# Autodesk Inventor assembly: SPE1V1 Estructura
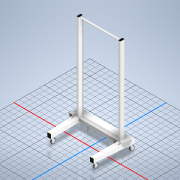
[picture p0: Inventor's stored thumbnail of the model, 180x180]
Saved by Autodesk Inventor 2021.2 (Build 252289000, 289)
## iProperties
Created: 2026-06-02
Part Number: SPE1V1 Estructura
Document SubType Name: Assembly
Designer: nelso
Author: nelso
## Documents named in this file (24)
- C:\Users\nelso\Documents\Escritorio\Soporte-Paciente-Espinografia\Workspace\SPE1V1 Estructura.iam
- C:\Users\nelso\Documents\Escritorio\Soporte-Paciente-Espinografia\Workspace\SP22V1 Tubo 40x80x1825mm.ipt
- C:\Users\nelso\Documents\Escritorio\Soporte-Paciente-Espinografia\Workspace\SP21V1 Tubo 40x80x100mm.ipt
- C:\Users\nelso\Documents\Escritorio\Soporte-Paciente-Espinografia\Workspace\SP23V1 Cobertora Derecha.ipt
- C:\Users\nelso\Documents\Escritorio\Soporte-Paciente-Espinografia\Workspace\SP24V1 Cobertora Izquierda.ipt
- C:\Users\nelso\Documents\Escritorio\Soporte-Paciente-Espinografia\Workspace\SP20V1 Tubo 80x120x790mm.ipt
- C:\Users\nelso\Documents\Escritorio\Soporte-Paciente-Espinografia\Workspace\SP19V1 Tapacanto Delantero.ipt
- C:\Users\nelso\Documents\Escritorio\Soporte-Paciente-Espinografia\Workspace\SP18V1 Tapacanto Superior.ipt
- C:\Users\nelso\Documents\Escritorio\Soporte-Paciente-Espinografia\Workspace\RFPLUS8PO300.ipt
- C:\Users\nelso\Documents\Escritorio\Soporte-Paciente-Espinografia\Workspace\SP17V1 Varilla Pedal.ipt
- C:\Users\nelso\Documents\Escritorio\Soporte-Paciente-Espinografia\Workspace\SP16V1 Buje Pedal.ipt
- C:\Users\nelso\Documents\Escritorio\Soporte-Paciente-Espinografia\Workspace\SP15V1 Pedal Izquierdo.ipt
- C:\Users\nelso\Documents\Escritorio\Soporte-Paciente-Espinografia\Workspace\SPE3V1 Freno.iam
- C:\Users\nelso\Documents\Escritorio\Soporte-Paciente-Espinografia\Workspace\SP14V1 Pedal Derecho.ipt
- C:\Users\nelso\Documents\Escritorio\Soporte-Paciente-Espinografia\Workspace\G3-100-PPP-RU.ipt
- C:\Users\nelso\Documents\Escritorio\Soporte-Paciente-Espinografia\Workspace\SP33V1 Tope Base.ipt
- C:\Users\nelso\Documents\Escritorio\Soporte-Paciente-Espinografia\Workspace\SP38V1 Cobertor Freno.ipt
- C:\Users\nelso\Documents\Escritorio\Soporte-Paciente-Espinografia\Workspace\SP43V1 Tubo 40x80x1825mm.ipt
- C:\Users\nelso\Documents\Escritorio\Soporte-Paciente-Espinografia\Workspace\DIN 555A10C.ipt
- C:\Users\nelso\Documents\Escritorio\Soporte-Paciente-Espinografia\Workspace\DIN125-A8,4C.ipt
- C:\Users\nelso\Documents\Escritorio\Soporte-Paciente-Espinografia\Workspace\DIN933M8X1.25L20C.ipt
- C:\Users\nelso\Documents\Escritorio\Soporte-Paciente-Espinografia\Workspace\SP11V1 Planchuela Baranda.ipt
- C:\Users\nelso\Documents\Escritorio\Soporte-Paciente-Espinografia\Workspace\SP52V1 Tubo superior.ipt
- C:\Users\nelso\Documents\Escritorio\Soporte-Paciente-Espinografia\Workspace\SP55V1 Chapa Guia.ipt
## Components (59 placed, 23 different names)
1. SP43V1 Tubo 40x80x1825mm:1 — Nivelación:17, Coincidencia:54, Coincidencia:55, Coincidencia:68, Nivelación:67, Coincidencia:71, Flush:75, Flush:76, Flush:77, Flush:78, Flush:79, Mate:84, Mate:85, Mate:86, Mate:87, Mate:88, Mate:107, Flush:101, Mate:235, Flush:149, Flush:150, Mate:238, Mate:239, Mate:242, Mate:246, Mate:247
2. SP18V1 Tapacanto Superior:1 — Coincidencia:68, Nivelación:67, Coincidencia:71
3. SP22V1 Tubo 40x80x1825mm:2 — Mate:179, Mate:180, Flush:120, Mate:181, Mate:182, Mate:183, Mate:184, Mate:185, Mate:186, Mate:187, Flush:121, Flush:122, Flush:123, Flush:124, Flush:125, Flush:126, Mate:222, Flush:145, Flush:146, Mate:236, Mate:237, Mate:243, Mate:244, Mate:245
4. SP18V1 Tapacanto Superior:2 — Mate:181
5. SP21V1 Tubo 40x80x100mm:1 — Nivelación:14, Coincidencia:24, Coincidencia:42, Mate:203, Mate:204, Flush:134
6. SP19V1 Tapacanto Delantero:1 — Mate:208, Flush:141, Flush:142
7. SP21V1 Tubo 40x80x100mm:2 — Coincidencia:37, Coincidencia:38, Coincidencia:66, Mate:206, Flush:136, Mate:207
8. SP21V1 Tubo 40x80x100mm:3 — Coincidencia:50, Coincidencia:51, Coincidencia:65, Mate:158, Mate:205, Flush:135
9. SP21V1 Tubo 40x80x100mm:4 — Mate:150, Mate:151, Mate:201, Mate:202, Flush:133
10. SP19V1 Tapacanto Delantero:2 — Flush:139, Flush:140, Mate:213
11. SP23V1 Cobertora Derecha:1 — Nivelación:14, Coincidencia:24, Nivelación:17, Coincidencia:37, Coincidencia:38, Nivelación:18, Coincidencia:42, Coincidencia:55, Nivelación:27, Coincidencia:66, Flush:105, Mate:126, Mate:131, Mate:174, Flush:118, Mate:194, Mate:195, Mate:196, Mate:197, Flush:131, Mate:208, Mate:210, Mate:212, Flush:141, Flush:142
12. SP24V1 Cobertora Izquierda:1 — Nivelación:18, Coincidencia:50, Coincidencia:51, Nivelación:24, Nivelación:28, Coincidencia:65, Flush:104, Mate:127, Mate:150, Mate:151, Mate:180, Flush:120, Mate:192, Mate:193, Mate:198, Mate:199, Flush:129, Mate:209, Flush:139, Flush:140, Mate:213
13. SP20V1 Tubo 80x120x790mm:1 — Nivelación:24, Coincidencia:54, Nivelación:27, Nivelación:28, Mate:110, Mate:111, Mate:124, Flush:119, Mate:177, Mate:179, Flush:127, Flush:137, Mate:209, Mate:210, Mate:211
14. RFPLUS8PO300:1 — Mate:107, Flush:101
15. RFPLUS8PO300:2 — Flush:75, Mate:88
16. RFPLUS8PO300:3 — Flush:76, Mate:87
17. RFPLUS8PO300:4 — Flush:77, Mate:86
18. RFPLUS8PO300:5 — Flush:78, Mate:84
19. RFPLUS8PO300:6 — Flush:79, Mate:85
20. SP17V1 Varilla Pedal:1 — Mate:117, Mate:118, Mate:119, Mate:120, Mate:121, Mate:125, Mate:128, Mate:129, Mate:130, Mate:132, Mate:133, Mate:134, Flush:127
21. SP16V1 Buje Pedal:1 — Mate:116, Flush:105, Mate:131
22. SP16V1 Buje Pedal:2 — Mate:116, Mate:125, Flush:104
23. SP14V1 Pedal Derecho:1 — Mate:128, Mate:129, Mate:130, Mate:132, Mate:200
24. SP15V1 Pedal Izquierdo:1 — Mate:120, Mate:121, Flush:132
25. SPE3V1 Freno:1 [sub-assembly] — Mate:110, Flush:103, Mate:117, Mate:118, Mate:119, Mate:124, Mate:127
26. SPE3V1 Freno:2 [sub-assembly] — Mate:111, Flush:103, Mate:126, Mate:133, Mate:134
27. RFPLUS8PO300:17 — Mate:187, Flush:121
28. RFPLUS8PO300:18 — Mate:186, Flush:122
29. RFPLUS8PO300:19 — Mate:185, Flush:123
30. RFPLUS8PO300:20 — Mate:184, Flush:124
31. RFPLUS8PO300:21 — Mate:182, Flush:125
32. RFPLUS8PO300:22 — Mate:183, Flush:126
33. G3-100-PPP-RU:1 — Mate:206, Flush:136, Mate:207
34. G3-100-PPP-RU:2 — Mate:203, Mate:204, Flush:134
35. G3-100-PPP-RU:3 — Mate:201, Mate:202, Flush:133
36. G3-100-PPP-RU:4 — Mate:158, Mate:205, Flush:135
37. SP33V1 Tope Base:1 — Mate:174, Flush:118, Mate:178
38. SP38V1 Cobertor Freno:1 — Flush:119, Mate:177, Mate:178, Flush:138
39. DIN 555A10C:1 — Mate:195, Mate:196
40. DIN 555A10C:2 — Mate:194, Mate:197
41. DIN 555A10C:3 — Mate:192, Mate:198
42. DIN 555A10C:4 — Mate:193, Mate:199
43. DIN125-A8,4C:1 — Mate:214, Mate:215, Mate:219
44. DIN933M8X1.25L20C:1 — Mate:214, Mate:215, Mate:220, Mate:224, Mate:236
45. SP11V1 Planchuela Baranda:1 — Mate:218, Mate:219, Mate:220, Mate:221, Mate:222
46. DIN125-A8,4C:2 — Mate:216, Mate:217, Mate:218
47. DIN933M8X1.25L20C:2 — Mate:216, Mate:217, Mate:221, Mate:223, Mate:237
48. RFPLUS8PO300:23 — Flush:146, Mate:223
49. RFPLUS8PO300:24 — Flush:145, Mate:224
50. DIN125-A8,4C:3
51. DIN933M8X1.25L20C:3 — Mate:238
52. SP11V1 Planchuela Baranda:2 — Mate:235, Mate:241
53. DIN125-A8,4C:4
54. DIN933M8X1.25L20C:4 — Mate:239
55. RFPLUS8PO300:25 — Flush:150
56. RFPLUS8PO300:26 — Flush:149
57. SP52V1 Tubo superior:1 — Mate:240, Mate:241
58. SP55V1 Chapa Guia:1 — Mate:243, Mate:244, Mate:245
59. SP55V1 Chapa Guia:2 — Mate:242, Mate:246, Mate:247
## Relationships (153: Mate 109, Flush 44)
- Nivelación:14 [Flush]: SP21V1 Tubo 40x80x100mm:1 ↔ SP23V1 Cobertora Derecha:1
- Coincidencia:24 [Mate] (0.5 mm): SP21V1 Tubo 40x80x100mm:1 ↔ SP23V1 Cobertora Derecha:1
- Nivelación:17 [Flush]: SP43V1 Tubo 40x80x1825mm:1 ↔ SP23V1 Cobertora Derecha:1
- Coincidencia:37 [Mate]: SP21V1 Tubo 40x80x100mm:2 ↔ SP23V1 Cobertora Derecha:1
- Coincidencia:38 [Mate]: SP21V1 Tubo 40x80x100mm:2 ↔ SP23V1 Cobertora Derecha:1
- Nivelación:18 [Flush]: SP23V1 Cobertora Derecha:1 ↔ SP24V1 Cobertora Izquierda:1
- Coincidencia:42 [Mate]: SP21V1 Tubo 40x80x100mm:1 ↔ SP23V1 Cobertora Derecha:1
- Coincidencia:50 [Mate]: SP21V1 Tubo 40x80x100mm:3 ↔ SP24V1 Cobertora Izquierda:1
- Coincidencia:51 [Mate]: SP21V1 Tubo 40x80x100mm:3 ↔ SP24V1 Cobertora Izquierda:1
- Nivelación:24 [Flush]: SP24V1 Cobertora Izquierda:1 ↔ SP20V1 Tubo 80x120x790mm:1
- Coincidencia:54 [Mate]: SP43V1 Tubo 40x80x1825mm:1 ↔ SP20V1 Tubo 80x120x790mm:1
- Coincidencia:55 [Mate]: SP43V1 Tubo 40x80x1825mm:1 ↔ SP23V1 Cobertora Derecha:1
- Nivelación:27 [Flush]: SP23V1 Cobertora Derecha:1 ↔ SP20V1 Tubo 80x120x790mm:1
- Nivelación:28 [Flush]: SP24V1 Cobertora Izquierda:1 ↔ SP20V1 Tubo 80x120x790mm:1
- Coincidencia:65 [Mate]: SP21V1 Tubo 40x80x100mm:3 ↔ SP24V1 Cobertora Izquierda:1
- Coincidencia:66 [Mate]: SP21V1 Tubo 40x80x100mm:2 ↔ SP23V1 Cobertora Derecha:1
- Coincidencia:68 [Mate]: SP43V1 Tubo 40x80x1825mm:1 ↔ SP18V1 Tapacanto Superior:1
- Nivelación:67 [Flush]: SP43V1 Tubo 40x80x1825mm:1 ↔ SP18V1 Tapacanto Superior:1
- Coincidencia:71 [Mate]: SP43V1 Tubo 40x80x1825mm:1 ↔ SP18V1 Tapacanto Superior:1
- Flush:75: SP43V1 Tubo 40x80x1825mm:1 ↔ RFPLUS8PO300:2
- Flush:76: SP43V1 Tubo 40x80x1825mm:1 ↔ RFPLUS8PO300:3
- Flush:77: SP43V1 Tubo 40x80x1825mm:1 ↔ RFPLUS8PO300:4
- Flush:78: SP43V1 Tubo 40x80x1825mm:1 ↔ RFPLUS8PO300:5
- Flush:79: SP43V1 Tubo 40x80x1825mm:1 ↔ RFPLUS8PO300:6
- Mate:84: SP43V1 Tubo 40x80x1825mm:1 ↔ RFPLUS8PO300:5
- Mate:85: SP43V1 Tubo 40x80x1825mm:1 ↔ RFPLUS8PO300:6
- Mate:86: SP43V1 Tubo 40x80x1825mm:1 ↔ RFPLUS8PO300:4
- Mate:87: SP43V1 Tubo 40x80x1825mm:1 ↔ RFPLUS8PO300:3
- Mate:88: SP43V1 Tubo 40x80x1825mm:1 ↔ RFPLUS8PO300:2
- Mate:107: SP43V1 Tubo 40x80x1825mm:1 ↔ RFPLUS8PO300:1
- Flush:101: SP43V1 Tubo 40x80x1825mm:1 ↔ RFPLUS8PO300:1
- Mate:110: SP20V1 Tubo 80x120x790mm:1 ↔ SPE3V1 Freno:1
- Mate:111: SP20V1 Tubo 80x120x790mm:1 ↔ SPE3V1 Freno:2
- Mate:116: SP16V1 Buje Pedal:1 ↔ SP16V1 Buje Pedal:2
- Flush:103: SPE3V1 Freno:1 ↔ SPE3V1 Freno:2
- Mate:117: SP17V1 Varilla Pedal:1 ↔ SPE3V1 Freno:1
- Mate:118: SP17V1 Varilla Pedal:1 ↔ SPE3V1 Freno:1
- Mate:119: SP17V1 Varilla Pedal:1 ↔ SPE3V1 Freno:1
- Mate:120: SP17V1 Varilla Pedal:1 ↔ SP15V1 Pedal Izquierdo:1
- Mate:121: SP17V1 Varilla Pedal:1 ↔ SP15V1 Pedal Izquierdo:1
- Mate:124: SP20V1 Tubo 80x120x790mm:1 ↔ SPE3V1 Freno:1
- Mate:125: SP17V1 Varilla Pedal:1 ↔ SP16V1 Buje Pedal:2
- Flush:104: SP24V1 Cobertora Izquierda:1 ↔ SP16V1 Buje Pedal:2
- Flush:105: SP23V1 Cobertora Derecha:1 ↔ SP16V1 Buje Pedal:1
- Mate:126 (100 mm): SP23V1 Cobertora Derecha:1 ↔ SPE3V1 Freno:2
- Mate:127 (100 mm): SP24V1 Cobertora Izquierda:1 ↔ SPE3V1 Freno:1
- Mate:128: SP17V1 Varilla Pedal:1 ↔ SP14V1 Pedal Derecho:1
- Mate:129: SP17V1 Varilla Pedal:1 ↔ SP14V1 Pedal Derecho:1
- Mate:130: SP17V1 Varilla Pedal:1 ↔ SP14V1 Pedal Derecho:1
- Mate:131: SP23V1 Cobertora Derecha:1 ↔ SP16V1 Buje Pedal:1
- Mate:132: SP17V1 Varilla Pedal:1 ↔ SP14V1 Pedal Derecho:1
- Mate:133: SP17V1 Varilla Pedal:1 ↔ SPE3V1 Freno:2
- Mate:134: SP17V1 Varilla Pedal:1 ↔ SPE3V1 Freno:2
- [Flush]: SP22V1 Tubo 40x80x1825mm:2 ↔ SP18V1 Tapacanto Superior:2
- [Mate]: SP22V1 Tubo 40x80x1825mm:2 ↔ SP18V1 Tapacanto Superior:2
- Mate:150 (0.5 mm): SP21V1 Tubo 40x80x100mm:4 ↔ SP24V1 Cobertora Izquierda:1
- Mate:151: SP21V1 Tubo 40x80x100mm:4 ↔ SP24V1 Cobertora Izquierda:1
- Mate:158: SP21V1 Tubo 40x80x100mm:3 ↔ G3-100-PPP-RU:4
- Mate:174: SP23V1 Cobertora Derecha:1 ↔ SP33V1 Tope Base:1
- Flush:118: SP23V1 Cobertora Derecha:1 ↔ SP33V1 Tope Base:1
- Flush:119: SP20V1 Tubo 80x120x790mm:1 ↔ SP38V1 Cobertor Freno:1
- Mate:177: SP20V1 Tubo 80x120x790mm:1 ↔ SP38V1 Cobertor Freno:1
- Mate:178: SP33V1 Tope Base:1 ↔ SP38V1 Cobertor Freno:1
- Mate:179: SP22V1 Tubo 40x80x1825mm:2 ↔ SP20V1 Tubo 80x120x790mm:1
- Mate:180: SP22V1 Tubo 40x80x1825mm:2 ↔ SP24V1 Cobertora Izquierda:1
- Flush:120: SP22V1 Tubo 40x80x1825mm:2 ↔ SP24V1 Cobertora Izquierda:1
- Mate:181: SP22V1 Tubo 40x80x1825mm:2 ↔ SP18V1 Tapacanto Superior:2
- Mate:182: SP22V1 Tubo 40x80x1825mm:2 ↔ RFPLUS8PO300:21
- Mate:183: SP22V1 Tubo 40x80x1825mm:2 ↔ RFPLUS8PO300:22
- Mate:184: SP22V1 Tubo 40x80x1825mm:2 ↔ RFPLUS8PO300:20
- Mate:185: SP22V1 Tubo 40x80x1825mm:2 ↔ RFPLUS8PO300:19
- Mate:186: SP22V1 Tubo 40x80x1825mm:2 ↔ RFPLUS8PO300:18
- Mate:187: SP22V1 Tubo 40x80x1825mm:2 ↔ RFPLUS8PO300:17
- Flush:121: SP22V1 Tubo 40x80x1825mm:2 ↔ RFPLUS8PO300:17
- Flush:122: SP22V1 Tubo 40x80x1825mm:2 ↔ RFPLUS8PO300:18
- Flush:123: SP22V1 Tubo 40x80x1825mm:2 ↔ RFPLUS8PO300:19
- Flush:124: SP22V1 Tubo 40x80x1825mm:2 ↔ RFPLUS8PO300:20
- Flush:125: SP22V1 Tubo 40x80x1825mm:2 ↔ RFPLUS8PO300:21
- Flush:126: SP22V1 Tubo 40x80x1825mm:2 ↔ RFPLUS8PO300:22
- Mate:192: SP24V1 Cobertora Izquierda:1 ↔ DIN 555A10C:3
- Mate:193: SP24V1 Cobertora Izquierda:1 ↔ DIN 555A10C:4
- Mate:194: SP23V1 Cobertora Derecha:1 ↔ DIN 555A10C:2
- Mate:195: SP23V1 Cobertora Derecha:1 ↔ DIN 555A10C:1
- Mate:196: SP23V1 Cobertora Derecha:1 ↔ DIN 555A10C:1
- Mate:197: SP23V1 Cobertora Derecha:1 ↔ DIN 555A10C:2
- Mate:198: SP24V1 Cobertora Izquierda:1 ↔ DIN 555A10C:3
- Mate:199: SP24V1 Cobertora Izquierda:1 ↔ DIN 555A10C:4
- Flush:127: SP20V1 Tubo 80x120x790mm:1 ↔ SP17V1 Varilla Pedal:1
- Flush:129 (7.5 mm): SP24V1 Cobertora Izquierda:1
- Flush:131 (7.5 mm): SP23V1 Cobertora Derecha:1
- Flush:132: SP15V1 Pedal Izquierdo:1
- Mate:200: SP14V1 Pedal Derecho:1
- Mate:201: SP21V1 Tubo 40x80x100mm:4 ↔ G3-100-PPP-RU:3
- Mate:202: SP21V1 Tubo 40x80x100mm:4 ↔ G3-100-PPP-RU:3
- Flush:133: SP21V1 Tubo 40x80x100mm:4 ↔ G3-100-PPP-RU:3
- Mate:203: SP21V1 Tubo 40x80x100mm:1 ↔ G3-100-PPP-RU:2
- Mate:204: SP21V1 Tubo 40x80x100mm:1 ↔ G3-100-PPP-RU:2
- Flush:134: SP21V1 Tubo 40x80x100mm:1 ↔ G3-100-PPP-RU:2
- Mate:205: SP21V1 Tubo 40x80x100mm:3 ↔ G3-100-PPP-RU:4
- Flush:135: SP21V1 Tubo 40x80x100mm:3 ↔ G3-100-PPP-RU:4
- Mate:206: SP21V1 Tubo 40x80x100mm:2 ↔ G3-100-PPP-RU:1
- Flush:136: SP21V1 Tubo 40x80x100mm:2 ↔ G3-100-PPP-RU:1
- Mate:207: SP21V1 Tubo 40x80x100mm:2 ↔ G3-100-PPP-RU:1
- Mate:208: SP19V1 Tapacanto Delantero:1 ↔ SP23V1 Cobertora Derecha:1
- Flush:137: SP20V1 Tubo 80x120x790mm:1
- Mate:209: SP24V1 Cobertora Izquierda:1 ↔ SP20V1 Tubo 80x120x790mm:1
- Mate:210: SP23V1 Cobertora Derecha:1 ↔ SP20V1 Tubo 80x120x790mm:1
- Mate:211: SP20V1 Tubo 80x120x790mm:1
- Flush:138: SP38V1 Cobertor Freno:1
- Mate:212 (380 mm): SP23V1 Cobertora Derecha:1
- Flush:139: SP19V1 Tapacanto Delantero:2 ↔ SP24V1 Cobertora Izquierda:1
- Flush:140: SP19V1 Tapacanto Delantero:2 ↔ SP24V1 Cobertora Izquierda:1
- Mate:213: SP19V1 Tapacanto Delantero:2 ↔ SP24V1 Cobertora Izquierda:1
- Flush:141: SP19V1 Tapacanto Delantero:1 ↔ SP23V1 Cobertora Derecha:1
- Flush:142: SP19V1 Tapacanto Delantero:1 ↔ SP23V1 Cobertora Derecha:1
- Mate:214: DIN125-A8,4C:1 ↔ DIN933M8X1.25L20C:1
- Mate:215: DIN125-A8,4C:1 ↔ DIN933M8X1.25L20C:1
- Mate:216: DIN125-A8,4C:2 ↔ DIN933M8X1.25L20C:2
- Mate:217: DIN125-A8,4C:2 ↔ DIN933M8X1.25L20C:2
- Mate:218: SP11V1 Planchuela Baranda:1 ↔ DIN125-A8,4C:2
- Mate:219: DIN125-A8,4C:1 ↔ SP11V1 Planchuela Baranda:1
- Mate:220: DIN933M8X1.25L20C:1 ↔ SP11V1 Planchuela Baranda:1
- Mate:221: SP11V1 Planchuela Baranda:1 ↔ DIN933M8X1.25L20C:2
- Mate:222: SP22V1 Tubo 40x80x1825mm:2 ↔ SP11V1 Planchuela Baranda:1
- Flush:145: SP22V1 Tubo 40x80x1825mm:2 ↔ RFPLUS8PO300:24
- Flush:146: SP22V1 Tubo 40x80x1825mm:2 ↔ RFPLUS8PO300:23
- Mate:223: DIN933M8X1.25L20C:2 ↔ RFPLUS8PO300:23
- Mate:224: DIN933M8X1.25L20C:1 ↔ RFPLUS8PO300:24
- [Mate]: DIN125-A8,4C:3 ↔ DIN933M8X1.25L20C:3
- [Mate]: DIN125-A8,4C:3 ↔ DIN933M8X1.25L20C:3
- [Mate]: DIN125-A8,4C:4 ↔ DIN933M8X1.25L20C:4
- [Mate]: DIN125-A8,4C:4 ↔ DIN933M8X1.25L20C:4
- [Mate]: SP11V1 Planchuela Baranda:2 ↔ DIN125-A8,4C:4
- [Mate]: DIN125-A8,4C:3 ↔ SP11V1 Planchuela Baranda:2
- [Mate]: DIN933M8X1.25L20C:3 ↔ SP11V1 Planchuela Baranda:2
- [Mate]: SP11V1 Planchuela Baranda:2 ↔ DIN933M8X1.25L20C:4
- [Mate]: DIN933M8X1.25L20C:4 ↔ RFPLUS8PO300:25
- [Mate]: DIN933M8X1.25L20C:3 ↔ RFPLUS8PO300:26
- Mate:235: SP43V1 Tubo 40x80x1825mm:1 ↔ SP11V1 Planchuela Baranda:2
- Flush:149: SP43V1 Tubo 40x80x1825mm:1 ↔ RFPLUS8PO300:26
- Flush:150: SP43V1 Tubo 40x80x1825mm:1 ↔ RFPLUS8PO300:25
- Mate:236: SP22V1 Tubo 40x80x1825mm:2 ↔ DIN933M8X1.25L20C:1
- Mate:237: SP22V1 Tubo 40x80x1825mm:2 ↔ DIN933M8X1.25L20C:2
- Mate:238: SP43V1 Tubo 40x80x1825mm:1 ↔ DIN933M8X1.25L20C:3
- Mate:239: SP43V1 Tubo 40x80x1825mm:1 ↔ DIN933M8X1.25L20C:4
- Mate:240: SP52V1 Tubo superior:1
- Mate:241: SP11V1 Planchuela Baranda:2 ↔ SP52V1 Tubo superior:1
- Mate:242: SP43V1 Tubo 40x80x1825mm:1 ↔ SP55V1 Chapa Guia:2
- Mate:243: SP22V1 Tubo 40x80x1825mm:2 ↔ SP55V1 Chapa Guia:1
- Mate:244: SP22V1 Tubo 40x80x1825mm:2 ↔ SP55V1 Chapa Guia:1
- Mate:245: SP22V1 Tubo 40x80x1825mm:2 ↔ SP55V1 Chapa Guia:1
- Mate:246: SP43V1 Tubo 40x80x1825mm:1 ↔ SP55V1 Chapa Guia:2
- Mate:247: SP43V1 Tubo 40x80x1825mm:1 ↔ SP55V1 Chapa Guia:2
## Named parameters: d314_d103 = 0 mm, d315_d104 = 0 mm, d464_d462 = 0 mm, d465_d463 = 0 mm, d466_d449 = 0 mm, d467_d450 = 0 mm, d468_d451 = 0 mm, d469_d452 = 0 mm, d470_d453 = 0 mm, d471_d454 = 0 mm, d472_d455 = 0 mm, d473_d456 = 0 mm
